# Autodesk Inventor assembly: Hopper roller rear assembly
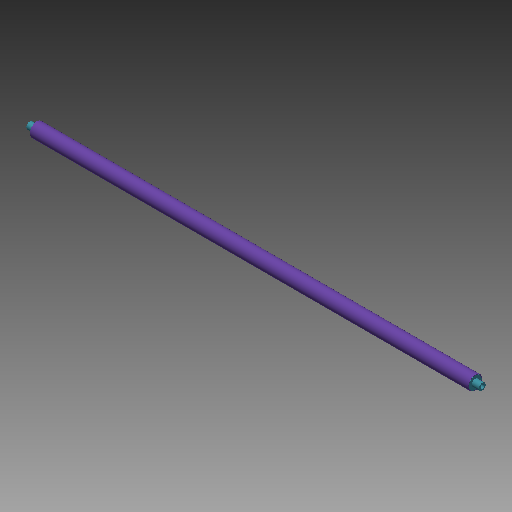
[picture p0: Inventor's stored thumbnail of the model, 512x512]
Saved by Autodesk Inventor 2017 (Build 210142000, 142)
## iProperties
Created: 2017-01-17
Part Number: Hopper roller rear assembly
Document SubType Name: Assembly
Designer: Ben
Author: Ben
## Documents named in this file (3)
- C:\Users\Ben\Desktop\Projects\2017 Robot\Ball Intake\Hopper roller rear assembly.iam
- C:\Users\Ben\Desktop\Projects\2017 Robot\Ball Intake\Hopper Roller Back.ipt
- C:\Users\Ben\Desktop\Projects\2017 Robot\Ball Intake\Hopper Roller Rear Plug.ipt
## Components (3 placed, 2 different names)
1. Hopper Roller Back:1 — Insert:1, Insert:2
2. Hopper Roller Rear Plug:1 — Insert:1
3. Hopper Roller Rear Plug:2 — Insert:2
## Relationships (2: Insert 2)
- Insert:1: Hopper Roller Back:1 ↔ Hopper Roller Rear Plug:1
- Insert:2: Hopper Roller Back:1 ↔ Hopper Roller Rear Plug:2
